# Autodesk Inventor assembly: CompleteRing
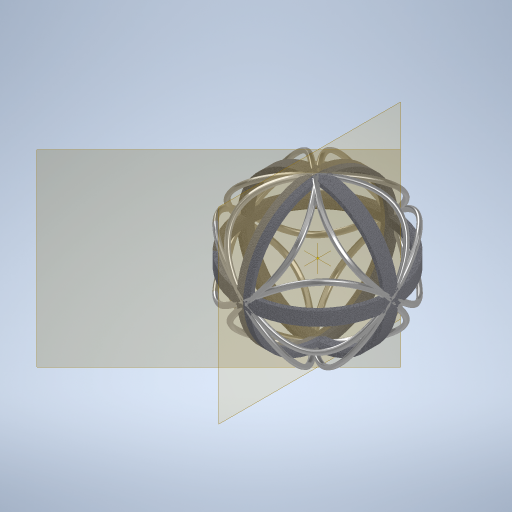
[picture p0: Inventor's stored thumbnail of the model, 512x512]
Saved by Autodesk Inventor 2023 (Build 270158000, 158)
## iProperties
Created: 2023-01-03
Part Number: CompleteRing
Document SubType Name: Assembly
Designer: redii
Author: redii
## Documents named in this file (6)
- C:\Users\redii\Desktop\CGM\My projectCube\OuterRing\CompleteRing.iam
- C:\Users\redii\Desktop\CGM\My projectCube\OuterRing\Ring.ipt
- C:\Users\redii\Desktop\CGM\My projectCube\OuterRing\RingSide1.ipt
- C:\Users\redii\Desktop\CGM\My projectCube\OuterRing\RingSide1_MIR.ipt
- C:\Users\redii\Desktop\CGM\My projectCube\OuterRing\RingSide1_MIR1.ipt
- C:\Users\redii\Desktop\CGM\My projectCube\OuterRing\RingSide1_MIR2.ipt
## Components (9 placed, 5 different names)
1. Ring:1 — Mate:7
2. Ring:2 — Mate:6
3. Ring:3
4. RingSide1:1 — Mate:20
5. RingSide1_MIR:1 — Mate:21
6. RingSide1:2 — Mate:22
7. RingSide1_MIR1:1 — Mate:23
8. RingSide1:3 — Mate:24
9. RingSide1_MIR2:1 — Mate:25
## Relationships (16: Mate 12, Angle 4)
- Mate:6: Ring:2
- Mate:7: Ring:1
- Mate:12
- Angle:1 (45 deg)
- Mate:13
- Angle:2 (45 deg)
- Mate:18
- Angle:3 (-45 deg)
- Mate:19
- Angle:4 (45 deg)
- Mate:20: RingSide1:1
- Mate:21: RingSide1_MIR:1
- Mate:22: RingSide1:2
- Mate:23: RingSide1_MIR1:1
- Mate:24: RingSide1:3
- Mate:25: RingSide1_MIR2:1
